# Autodesk Inventor assembly: 関節3
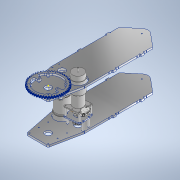
[picture p0: Inventor's stored thumbnail of the model, 180x180]
Saved by Autodesk Inventor 2021 (Build 250183000, 183)
## iProperties
Created: 2022-02-01
Part Number: 関節3
Document SubType Name: Assembly
Designer: hirohumi
Author: hirohumi
## Documents named in this file (18)
- C:\Users\hirohumi\OneDrive\ドキュメント\ロボ研\2022NHKロボコン\R2_version1\3軸アーム\関節3.iam
- C:\Users\hirohumi\OneDrive\ドキュメント\ロボ研\2022NHKロボコン\R2_version1\3軸アーム\ギア_歯数50.ipt
- C:\Users\hirohumi\OneDrive\ドキュメント\ロボ研\2022NHKロボコン\R2_version1\3軸アーム\関節3_775側_プーリ側板.ipt
- C:\Users\hirohumi\OneDrive\ドキュメント\ロボ研\2022NHKロボコン\R2_version1\3軸アーム\軸6-25.ipt
- C:\Users\hirohumi\OneDrive\ドキュメント\ロボ研\2022NHKロボコン\R2_version1\3軸アーム\関節3_775側_モータマウント.ipt
- C:\Users\hirohumi\OneDrive\ドキュメント\ロボ研\2022NHKロボコン\R2_version1\RS-775GM104 v1.ipt
- C:\Users\hirohumi\OneDrive\ドキュメント\ロボ研\2022NHKロボコン\R2_version1\3軸アーム\カップリング_軸8mm.ipt
- C:\Users\hirohumi\OneDrive\ドキュメント\ロボ研\2022NHKロボコン\R2_version1\3軸アーム\カップリング_軸8mm_2.5mm.ipt
- C:\Users\hirohumi\OneDrive\ドキュメント\ロボ研\2022NHKロボコン\R2_version1\3軸アーム\軸6-5.ipt
- C:\Users\hirohumi\OneDrive\ドキュメント\ロボ研\2022NHKロボコン\R2_version1\3軸アーム\関節3_555側_モータマウント.ipt
- C:\Users\hirohumi\OneDrive\ドキュメント\ロボ研\2022NHKロボコン\R2_version1\RS-555-71.ipt
- C:\Users\hirohumi\OneDrive\ドキュメント\ロボ研\2022NHKロボコン\R2_version1\3軸アーム\カップリング_軸6mm.ipt
- C:\Users\hirohumi\OneDrive\ドキュメント\ロボ研\2022NHKロボコン\R2_version1\3軸アーム\軸8-30.ipt
- C:\Users\hirohumi\OneDrive\ドキュメント\ロボ研\2022NHKロボコン\R2_version1\3軸アーム\プーリ_歯数15.ipt
- C:\Users\hirohumi\OneDrive\ドキュメント\ロボ研\2022NHKロボコン\R2_version1\3軸アーム\プーリ_歯数15_2.5mm.ipt
- C:\Users\hirohumi\OneDrive\ドキュメント\ロボ研\2022NHKロボコン\R2_version1\3軸アーム\AMT102Normal\CUI_DEVICES_AMT102-0048-N8000-S.iam
- C:\Users\hirohumi\OneDrive\ドキュメント\ロボ研\2022NHKロボコン\R2_version1\3軸アーム\エンコーダマウント.ipt
- C:\Users\hirohumi\OneDrive\ドキュメント\ロボ研\2022NHKロボコン\R2_version1\3軸アーム\関節3_側板3.ipt
## Components (43 placed, 17 different names)
1. 関節3_775側_プーリ側板:1 — 挿入:9, 挿入:10, 挿入:11, 挿入:12, 挿入:66, 挿入:67, 挿入:82, 挿入:83
2. 軸6-25:1 — 挿入:9
3. 軸6-25:2 — 挿入:10, 挿入:13
4. 軸6-25:3 — 挿入:11, 挿入:14
5. 軸6-25:4 — 挿入:12
6. 関節3_775側_モータマウント:1 — 挿入:13, 挿入:14, 挿入:15, 挿入:16, 挿入:70, 挿入:71
7. RS-775GM104 v1:1 — 挿入:15, 挿入:16, 挿入:19, メイト:4
8. カップリング_軸8mm:1 — 挿入:17, 挿入:18
9. カップリング_軸8mm_2.5mm:1 — 挿入:17, 挿入:18, 挿入:19, 挿入:51
10. 軸6-5:1 — 挿入:26, 挿入:90
11. 軸6-5:3 — 挿入:27, 挿入:91
12. ギア_歯数50:1 — 挿入:26, 挿入:27
13. 関節3_775側_プーリ側板:2 — 挿入:40, 挿入:41, 挿入:42, 挿入:43, 挿入:76, 挿入:77, 挿入:84, 挿入:85
14. 軸6-25:5 — 挿入:40, 挿入:44
15. 軸6-25:6 — 挿入:41
16. 軸6-25:7 — 挿入:42, 挿入:45
17. 軸6-25:8 — 挿入:43
18. 関節3_555側_モータマウント:1 — 挿入:44, 挿入:45, 挿入:46, 挿入:47, 挿入:80, 挿入:81
19. RS-555-71:1 — 挿入:46, 挿入:47, 挿入:50
20. カップリング_軸6mm:1 — 挿入:48, 挿入:49, 挿入:50, 挿入:52
21. カップリング_軸8mm_2.5mm:2 — 挿入:48, 挿入:49
22. 軸8-30:1 — 挿入:51, メイト:1
23. 軸8-30:2 — 挿入:52, メイト:2
24. プーリ_歯数15:1 — 挿入:54, 挿入:55, 挿入:56, 挿入:57
25. プーリ_歯数15_2.5mm:1 — 挿入:54, 挿入:55
26. カップリング_軸8mm:2 — 挿入:56, 挿入:57, メイト:2
27. プーリ_歯数15:2
28. プーリ_歯数15_2.5mm:2
29. カップリング_軸8mm:3 — メイト:1
30. 軸6-25:9 — 挿入:83
31. 軸6-25:10 — 挿入:66
32. 軸6-25:11 — 挿入:67, 挿入:87
33. 軸6-25:12 — 挿入:82, 挿入:86
34. 軸6-25:13 — 挿入:76, 挿入:88
35. 軸6-25:14 — 挿入:85
36. 軸6-25:15 — 挿入:84
37. 軸6-25:16 — 挿入:77, 挿入:89
38. CUI_DEVICES_AMT102-0048-N8000-S:1 [sub-assembly] — 挿入:68, 挿入:69
39. CUI_DEVICES_AMT102-0048-N8000-S:2 [sub-assembly] — 挿入:78, 挿入:79
40. エンコーダマウント:1 — 挿入:68, 挿入:69, 挿入:70, 挿入:71
41. エンコーダマウント:2 — 挿入:78, 挿入:79, 挿入:80, 挿入:81
42. 関節3_側板3:1 — 挿入:86, 挿入:87, メイト:3, 挿入:90, 挿入:91
43. 関節3_側板3:2 — 挿入:88, 挿入:89, メイト:3, メイト:4
## Relationships (60: Insert 56, Mate 4)
- 挿入:9 [Insert]: 関節3_775側_プーリ側板:1 ↔ 軸6-25:1
- 挿入:10 [Insert]: 関節3_775側_プーリ側板:1 ↔ 軸6-25:2
- 挿入:11 [Insert]: 関節3_775側_プーリ側板:1 ↔ 軸6-25:3
- 挿入:12 [Insert]: 関節3_775側_プーリ側板:1 ↔ 軸6-25:4
- 挿入:13 [Insert]: 軸6-25:2 ↔ 関節3_775側_モータマウント:1
- 挿入:14 [Insert]: 軸6-25:3 ↔ 関節3_775側_モータマウント:1
- 挿入:15 [Insert]: 関節3_775側_モータマウント:1 ↔ RS-775GM104 v1:1
- 挿入:16 [Insert]: 関節3_775側_モータマウント:1 ↔ RS-775GM104 v1:1
- 挿入:17 [Insert]: カップリング_軸8mm:1 ↔ カップリング_軸8mm_2.5mm:1
- 挿入:18 [Insert]: カップリング_軸8mm:1 ↔ カップリング_軸8mm_2.5mm:1
- 挿入:19 [Insert]: RS-775GM104 v1:1 ↔ カップリング_軸8mm_2.5mm:1
- 挿入:26 [Insert]: 軸6-5:1 ↔ ギア_歯数50:1
- 挿入:27 [Insert]: 軸6-5:3 ↔ ギア_歯数50:1
- 挿入:40 [Insert]: 関節3_775側_プーリ側板:2 ↔ 軸6-25:5
- 挿入:41 [Insert]: 関節3_775側_プーリ側板:2 ↔ 軸6-25:6
- 挿入:42 [Insert]: 関節3_775側_プーリ側板:2 ↔ 軸6-25:7
- 挿入:43 [Insert]: 関節3_775側_プーリ側板:2 ↔ 軸6-25:8
- 挿入:44 [Insert]: 軸6-25:5 ↔ 関節3_555側_モータマウント:1
- 挿入:45 [Insert]: 軸6-25:7 ↔ 関節3_555側_モータマウント:1
- 挿入:46 [Insert]: 関節3_555側_モータマウント:1 ↔ RS-555-71:1
- 挿入:47 [Insert]: 関節3_555側_モータマウント:1 ↔ RS-555-71:1
- 挿入:48 [Insert]: カップリング_軸6mm:1 ↔ カップリング_軸8mm_2.5mm:2
- 挿入:49 [Insert]: カップリング_軸6mm:1 ↔ カップリング_軸8mm_2.5mm:2
- 挿入:50 [Insert]: RS-555-71:1 ↔ カップリング_軸6mm:1
- 挿入:51 [Insert]: カップリング_軸8mm_2.5mm:1 ↔ 軸8-30:1
- 挿入:52 [Insert]: カップリング_軸6mm:1 ↔ 軸8-30:2
- 挿入:54 [Insert]: プーリ_歯数15:1 ↔ プーリ_歯数15_2.5mm:1
- 挿入:55 [Insert]: プーリ_歯数15:1 ↔ プーリ_歯数15_2.5mm:1
- 挿入:56 [Insert]: プーリ_歯数15:1 ↔ カップリング_軸8mm:2
- 挿入:57 [Insert]: プーリ_歯数15:1 ↔ カップリング_軸8mm:2
- [Insert]: プーリ_歯数15:2 ↔ プーリ_歯数15_2.5mm:2
- [Insert]: プーリ_歯数15:2 ↔ プーリ_歯数15_2.5mm:2
- [Insert]: プーリ_歯数15:2 ↔ カップリング_軸8mm:3
- [Insert]: プーリ_歯数15:2 ↔ カップリング_軸8mm:3
- メイト:1 [Mate]: 軸8-30:1 ↔ カップリング_軸8mm:3
- メイト:2 [Mate]: 軸8-30:2 ↔ カップリング_軸8mm:2
- 挿入:66 [Insert]: 関節3_775側_プーリ側板:1 ↔ 軸6-25:10
- 挿入:67 [Insert]: 関節3_775側_プーリ側板:1 ↔ 軸6-25:11
- 挿入:68 [Insert]: CUI_DEVICES_AMT102-0048-N8000-S:1 ↔ エンコーダマウント:1
- 挿入:69 [Insert]: CUI_DEVICES_AMT102-0048-N8000-S:1 ↔ エンコーダマウント:1
- 挿入:70 [Insert]: 関節3_775側_モータマウント:1 ↔ エンコーダマウント:1
- 挿入:71 [Insert]: 関節3_775側_モータマウント:1 ↔ エンコーダマウント:1
- 挿入:76 [Insert]: 関節3_775側_プーリ側板:2 ↔ 軸6-25:13
- 挿入:77 [Insert]: 関節3_775側_プーリ側板:2 ↔ 軸6-25:16
- 挿入:78 [Insert]: CUI_DEVICES_AMT102-0048-N8000-S:2 ↔ エンコーダマウント:2
- 挿入:79 [Insert]: CUI_DEVICES_AMT102-0048-N8000-S:2 ↔ エンコーダマウント:2
- 挿入:80 [Insert]: 関節3_555側_モータマウント:1 ↔ エンコーダマウント:2
- 挿入:81 [Insert]: 関節3_555側_モータマウント:1 ↔ エンコーダマウント:2
- 挿入:82 [Insert]: 関節3_775側_プーリ側板:1 ↔ 軸6-25:12
- 挿入:83 [Insert]: 関節3_775側_プーリ側板:1 ↔ 軸6-25:9
- 挿入:84 [Insert]: 関節3_775側_プーリ側板:2 ↔ 軸6-25:15
- 挿入:85 [Insert]: 関節3_775側_プーリ側板:2 ↔ 軸6-25:14
- 挿入:86 [Insert]: 軸6-25:12 ↔ 関節3_側板3:1
- 挿入:87 [Insert]: 軸6-25:11 ↔ 関節3_側板3:1
- 挿入:88 [Insert]: 軸6-25:13 ↔ 関節3_側板3:2
- 挿入:89 [Insert]: 軸6-25:16 ↔ 関節3_側板3:2
- メイト:3 [Mate]: 関節3_側板3:1 ↔ 関節3_側板3:2
- 挿入:90 [Insert]: 軸6-5:1 ↔ 関節3_側板3:1
- 挿入:91 [Insert]: 軸6-5:3 ↔ 関節3_側板3:1
- メイト:4 [Mate]: RS-775GM104 v1:1 ↔ 関節3_側板3:2
## Named parameters: d57_d55 = 0 mm, d58_d56 = 0 mm, d59_d53 = 0 mm, d60_d54 = 0 mm
